# Autodesk Inventor assembly: Robot Assembly
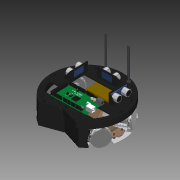
[picture p0: Inventor's stored thumbnail of the model, 180x180]
Saved by Autodesk Inventor 2015 (Build 190159000, 159)
## iProperties
Created: 2015-10-10
Part Number: Robot Assembly
Document SubType Name: Assembly
Designer: James
Mass: 1382.52 g
Surface Area: 3536.41 cm^2
Volume: 667.036 cm^3
Density: 2.07263 g/cm^3
Author: James
## Documents named in this file (21)
- C:\Users\James\Dropbox\Robotics 2016\Design\3D Printing\Robot Assembly.iam
- C:\Users\James\Dropbox\Robotics 2016\Design\3D Printing\Bottom Plate.ipt
- C:\Users\James\Dropbox\Robotics 2016\Design\3D Printing\Rod.ipt
- C:\Users\James\Dropbox\Robotics 2016\Design\3D Printing\Bottom Plate Standoff.ipt
- C:\Users\James\Dropbox\Robotics 2016\Design\3D Printing\Motor Mount Standoff.ipt
- C:\Users\James\Dropbox\Robotics 2016\Design\3D Printing\Motor Mount Bracket.ipt
- C:\Users\James\Dropbox\Robotics 2016\Design\3D Printing\Motor.ipt
- C:\Users\James\Dropbox\Robotics 2016\Design\3D Printing\Spacer 5.ipt
- C:\Users\James\Dropbox\Robotics 2016\Design\3D Printing\Veroboard Bottom Plate.ipt
- C:\Users\James\Dropbox\Robotics 2016\Design\3D Printing\Rod Spacer.ipt
- C:\Users\James\Dropbox\Robotics 2016\Design\3D Printing\Middle Plate.ipt
- C:\Users\James\Dropbox\Robotics 2016\Design\3D Printing\Nut Rod.ipt
- C:\Users\James\Dropbox\Robotics 2016\Design\3D Printing\Wheel.ipt
- C:\Users\James\Dropbox\Robotics 2016\Design\3D Printing\ArduinoMEGA2560.ipt
- C:\Users\James\Dropbox\Robotics 2016\Design\3D Printing\Verboard Middle Plate.ipt
- C:\Users\James\Dropbox\Robotics 2016\Design\3D Printing\M3 6mm screw.ipt
- C:\Users\James\Dropbox\Robotics 2016\Design\3D Printing\M3 hex nut.ipt
- C:\Users\James\Dropbox\Robotics 2016\Design\3D Printing\HC-SR04 Sonar.ipt
- C:\Users\James\Dropbox\Robotics 2016\Design\3D Printing\Battery.ipt
- C:\Users\James\Dropbox\Robotics 2016\Design\3D Printing\Spacer 25.ipt
- C:\Users\James\Dropbox\Robotics 2016\Design\3D Printing\Spacer 45.ipt
## Components (99 placed, 20 different names)
1. Bottom Plate:1 — Mate:2, Mate:3, Mate:5, Mate:6, Mate:9, Mate:12, Mate:13, Mate:14, Mate:15, Mate:16, Mate:17, Mate:18, Mate:19, Mate:20, Mate:21, Mate:22, Mate:23, Mate:48, Mate:49, Mate:50, Mate:51, Mate:52, Mate:53, Mate:54, Mate:55, Mate:56, Mate:57, Mate:58, Mate:59, Mate:60, Mate:61, Mate:62, Mate:63, Mate:64, Mate:65, Mate:66, Mate:67, Mate:68, Mate:69, Mate:70, Mate:71, Mate:72, Mate:73, Mate:74, Mate:75, Mate:153, Mate:154, Mate:155, Mate:156, Mate:157, Mate:158, Mate:159, Mate:160, Mate:161, Mate:162, Mate:163, Mate:164, Mate:165, Mate:166, Mate:167, Mate:168, Mate:169, Mate:170, Mate:171, Mate:172, Mate:173, Mate:174, Mate:175, Mate:176, Mate:177, Mate:178, Mate:179, Mate:180, Mate:381, Mate:382, Mate:385, Mate:386, Mate:387, Mate:388, Mate:389, Mate:390, Mate:443, Mate:444
2. Rod:2 — Mate:2, Mate:6, Mate:91, Mate:384
3. Rod:3 — Mate:3, Mate:5, Mate:90, Mate:383
4. Bottom Plate Standoff:1 — Mate:9, Mate:83
5. Motor Mount Standoff:1 — Mate:12, Mate:20, Mate:21, Mate:24, Mate:32, Mate:33
6. Motor Mount Standoff:2 — Mate:13, Mate:16, Mate:17, Mate:25, Mate:30, Mate:31
7. Motor Mount Standoff:3 — Mate:14, Mate:22, Mate:23, Mate:26, Mate:34, Mate:35
8. Motor Mount Standoff:4 — Mate:15, Mate:18, Mate:19, Mate:27, Mate:28, Mate:29
9. Motor Mount Bracket:1 — Mate:25, Mate:30, Mate:31, Mate:37, Mate:41, Mate:46
10. Motor Mount Bracket:2 — Mate:27, Mate:28, Mate:29, Mate:39, Mate:42, Mate:47
11. Motor Mount Bracket:3 — Mate:26, Mate:34, Mate:35, Mate:38, Mate:40, Mate:45
12. Motor Mount Bracket:4 — Mate:24, Mate:32, Mate:33, Mate:36, Mate:43, Mate:44
13. Motor:1 — Mate:36, Mate:43, Mate:44, Flush:4, Mate:97
14. Motor:2 — Mate:37, Mate:41, Mate:46, Flush:1, Mate:94
15. Motor:3 — Mate:38, Mate:40, Mate:45, Flush:3, Mate:96
16. Motor:4 — Mate:39, Mate:42, Mate:47, Flush:2, Mate:95
17. Spacer 5:1 — Mate:53, Mate:69, Mate:204
18. Spacer 5:2 — Mate:52, Mate:73, Mate:205
19. Spacer 5:3 — Mate:49, Mate:68, Mate:420
20. Spacer 5:4 — Mate:48, Mate:67, Mate:77, Mate:425
21. Spacer 5:5 — Mate:51, Mate:64, Mate:76, Mate:421
22. Spacer 5:6 — Mate:50, Mate:65, Mate:423
23. Spacer 5:7 — Mate:55, Mate:62, Mate:195
24. Spacer 5:8 — Mate:54, Mate:66, Mate:78, Mate:427
25. Spacer 5:9 — Mate:56, Mate:71, Mate:200
26. Spacer 5:10 — Mate:57, Mate:74, Mate:201
27. Spacer 5:11 — Mate:60, Mate:75, Mate:206
28. Spacer 5:12 — Mate:58, Mate:63, Mate:196
29. Spacer 5:13 — Mate:59, Mate:72, Mate:202
30. Spacer 5:14 — Mate:61, Mate:70, Mate:199
31. Veroboard Bottom Plate:1 — Mate:76, Mate:77, Mate:78, Mate:181, Mate:183, Mate:184, Mate:185, Mate:186, Mate:187, Mate:188, Mate:189, Mate:191, Mate:193, Mate:422, Mate:424, Mate:426, Mate:428
32. Rod Spacer:1 — Mate:382, Mate:383, Mate:385, Mate:391, Mate:395, Mate:396
33. Rod Spacer:2 — Mate:381, Mate:384, Mate:386, Mate:393, Mate:397
34. Middle Plate:1 — Mate:83, Mate:86, Mate:89, Mate:109, Mate:111, Mate:113, Mate:114, Mate:116, Mate:221, Mate:222, Mate:223, Mate:224, Mate:225, Mate:250, Mate:251, Mate:375, Mate:376, Mate:377, Mate:378, Mate:379, Mate:380, Mate:399, Mate:401, Mate:402, Mate:440, Mate:441, Mate:442
35. Nut Rod:1 — Mate:86, Mate:91
36. Nut Rod:4 — Mate:89, Mate:90
37. Wheel:1 — Flush:4, Mate:97
38. Wheel:2 — Flush:3, Mate:96
39. Wheel:3 — Flush:2, Mate:95
40. Wheel:4 — Flush:1, Mate:94
41. Spacer 5:15 — Mate:114, Mate:225, Mate:226, Mate:257
42. Spacer 5:17 — Mate:111, Mate:221, Mate:227, Mate:243
43. Spacer 5:20 — Mate:109, Mate:223, Mate:247
44. Spacer 5:22 — Mate:113, Mate:222, Mate:242
45. Spacer 5:23 — Mate:116, Mate:224, Mate:228, Mate:256
46. -  -:1 — Mate:226, Mate:227, Mate:228, Mate:229, Mate:230, Mate:231, Mate:232, Mate:233, Mate:234, Mate:235, Mate:236, Mate:237, Mate:238
47. Verboard Middle Plate:1 — Mate:429, Mate:430, Mate:431, Mate:432, Mate:433, Mate:434, Mate:435
48. M3 6mm screw:6 — Mate:153, Mate:165
49. M3 6mm screw:8 — Mate:154, Mate:167
50. M3 6mm screw:9 — Mate:155, Mate:168
51. M3 6mm screw:10 — Mate:156, Mate:170
52. M3 6mm screw:11 — Mate:157, Mate:166
53. M3 6mm screw:12 — Mate:158, Mate:171
54. M3 6mm screw:13 — Mate:159, Mate:172
55. M3 6mm screw:14 — Mate:160, Mate:169
56. M3 6mm screw:15 — Mate:161, Mate:173
57. M3 6mm screw:16 — Mate:162, Mate:174
58. M3 6mm screw:17 — Mate:163, Mate:175
59. M3 6mm screw:18 — Mate:164, Mate:176
60. M3 6mm screw:19 — Mate:177, Mate:179
61. M3 6mm screw:20 — Mate:178, Mate:180
62. M3 hex nut:1 — Mate:181, Mate:196
63. M3 hex nut:3 — Mate:183, Mate:204
64. M3 hex nut:4 — Mate:184, Mate:200
65. M3 hex nut:5 — Mate:185, Mate:202
66. M3 hex nut:6 — Mate:186, Mate:205
67. M3 hex nut:7 — Mate:188, Mate:206
68. M3 hex nut:8 — Mate:187, Mate:420
69. M3 hex nut:9 — Mate:189, Mate:195
70. M3 hex nut:11 — Mate:193, Mate:199
71. M3 hex nut:12 — Mate:191, Mate:201
72. M3 hex nut:15 — Mate:247, Mate:402
73. M3 hex nut:17 — Mate:242, Mate:401
74. M3 hex nut:21 — Mate:243, Mate:399
75. M3 6mm screw:21 — Mate:230, Mate:234
76. M3 6mm screw:22 — Mate:233, Mate:237
77. M3 6mm screw:23 — Mate:232, Mate:238
78. M3 6mm screw:24 — Mate:231, Mate:235
79. M3 6mm screw:25 — Mate:229, Mate:236
80. M3 hex nut:26 — Mate:251, Mate:256
81. M3 hex nut:27 — Mate:250, Mate:257
82. HC-SR04 Sonar:1 — Mate:375, Mate:376, Mate:377
83. HC-SR04 Sonar:2 — Mate:378, Mate:379, Mate:380
84. Battery:1 — Mate:395, Mate:396, Mate:397
85. M3 6mm screw:34 — Mate:387, Mate:389, Mate:394
86. M3 6mm screw:35 — Mate:388, Mate:390, Mate:392
87. M3 hex nut:32 — Mate:391, Mate:392
88. M3 hex nut:33 — Mate:393, Mate:394
89. Spacer 25:1 — Mate:427, Mate:428, Mate:430, Mate:439
90. Spacer 25:2 — Mate:425, Mate:426, Mate:431, Mate:438
91. Spacer 25:3 — Mate:423, Mate:424, Mate:437
92. Spacer 25:4 — Mate:421, Mate:422, Mate:429, Mate:436
93. M3 hex nut:34 — Mate:434, Mate:437
94. M3 hex nut:35 — Mate:435, Mate:439
95. M3 hex nut:36 — Mate:433, Mate:436
96. M3 hex nut:37 — Mate:432, Mate:438
97. HC-SR04 Sonar:3 — Mate:440, Mate:441, Mate:442
98. Spacer 45:1 — Mate:443, Mate:444
99. Spacer 45:2
## Relationships (213: Mate 209, Flush 4)
- Mate:2: Bottom Plate:1 ↔ Rod:2
- Mate:3: Bottom Plate:1 ↔ Rod:3
- Mate:5: Bottom Plate:1 ↔ Rod:3
- Mate:6: Bottom Plate:1 ↔ Rod:2
- Mate:9: Bottom Plate:1 ↔ Bottom Plate Standoff:1
- Mate:12: Bottom Plate:1 ↔ Motor Mount Standoff:1
- Mate:13: Bottom Plate:1 ↔ Motor Mount Standoff:2
- Mate:14: Bottom Plate:1 ↔ Motor Mount Standoff:3
- Mate:15: Bottom Plate:1 ↔ Motor Mount Standoff:4
- Mate:16: Bottom Plate:1 ↔ Motor Mount Standoff:2
- Mate:17: Bottom Plate:1 ↔ Motor Mount Standoff:2
- Mate:18: Bottom Plate:1 ↔ Motor Mount Standoff:4
- Mate:19: Bottom Plate:1 ↔ Motor Mount Standoff:4
- Mate:20: Bottom Plate:1 ↔ Motor Mount Standoff:1
- Mate:21: Bottom Plate:1 ↔ Motor Mount Standoff:1
- Mate:22: Bottom Plate:1 ↔ Motor Mount Standoff:3
- Mate:23: Bottom Plate:1 ↔ Motor Mount Standoff:3
- Mate:24: Motor Mount Standoff:1 ↔ Motor Mount Bracket:4
- Mate:25: Motor Mount Standoff:2 ↔ Motor Mount Bracket:1
- Mate:26: Motor Mount Standoff:3 ↔ Motor Mount Bracket:3
- Mate:27: Motor Mount Standoff:4 ↔ Motor Mount Bracket:2
- Mate:28: Motor Mount Standoff:4 ↔ Motor Mount Bracket:2
- Mate:29: Motor Mount Standoff:4 ↔ Motor Mount Bracket:2
- Mate:30: Motor Mount Standoff:2 ↔ Motor Mount Bracket:1
- Mate:31: Motor Mount Standoff:2 ↔ Motor Mount Bracket:1
- Mate:32: Motor Mount Standoff:1 ↔ Motor Mount Bracket:4
- Mate:33: Motor Mount Standoff:1 ↔ Motor Mount Bracket:4
- Mate:34: Motor Mount Standoff:3 ↔ Motor Mount Bracket:3
- Mate:35: Motor Mount Standoff:3 ↔ Motor Mount Bracket:3
- Mate:36: Motor Mount Bracket:4 ↔ Motor:1
- Mate:37: Motor Mount Bracket:1 ↔ Motor:2
- Mate:38: Motor Mount Bracket:3 ↔ Motor:3
- Mate:39: Motor Mount Bracket:2 ↔ Motor:4
- Mate:40: Motor Mount Bracket:3 ↔ Motor:3
- Mate:41: Motor Mount Bracket:1 ↔ Motor:2
- Mate:42: Motor Mount Bracket:2 ↔ Motor:4
- Mate:43: Motor Mount Bracket:4 ↔ Motor:1
- Mate:44: Motor Mount Bracket:4 ↔ Motor:1
- Mate:45: Motor Mount Bracket:3 ↔ Motor:3
- Mate:46: Motor Mount Bracket:1 ↔ Motor:2
- Mate:47: Motor Mount Bracket:2 ↔ Motor:4
- Mate:48: Bottom Plate:1 ↔ Spacer 5:4
- Mate:49: Bottom Plate:1 ↔ Spacer 5:3
- Mate:50: Bottom Plate:1 ↔ Spacer 5:6
- Mate:51: Bottom Plate:1 ↔ Spacer 5:5
- Mate:52: Bottom Plate:1 ↔ Spacer 5:2
- Mate:53: Bottom Plate:1 ↔ Spacer 5:1
- Mate:54: Bottom Plate:1 ↔ Spacer 5:8
- Mate:55: Bottom Plate:1 ↔ Spacer 5:7
- Mate:56: Bottom Plate:1 ↔ Spacer 5:9
- Mate:57: Bottom Plate:1 ↔ Spacer 5:10
- Mate:58: Bottom Plate:1 ↔ Spacer 5:12
- Mate:59: Bottom Plate:1 ↔ Spacer 5:13
- Mate:60: Bottom Plate:1 ↔ Spacer 5:11
- Mate:61: Bottom Plate:1 ↔ Spacer 5:14
- Mate:62: Bottom Plate:1 ↔ Spacer 5:7
- Mate:63: Bottom Plate:1 ↔ Spacer 5:12
- Mate:64: Bottom Plate:1 ↔ Spacer 5:5
- Mate:65: Bottom Plate:1 ↔ Spacer 5:6
- Mate:66: Bottom Plate:1 ↔ Spacer 5:8
- Mate:67: Bottom Plate:1 ↔ Spacer 5:4
- Mate:68: Bottom Plate:1 ↔ Spacer 5:3
- Mate:69: Bottom Plate:1 ↔ Spacer 5:1
- Mate:70: Bottom Plate:1 ↔ Spacer 5:14
- Mate:71: Bottom Plate:1 ↔ Spacer 5:9
- Mate:72: Bottom Plate:1 ↔ Spacer 5:13
- Mate:73: Bottom Plate:1 ↔ Spacer 5:2
- Mate:74: Bottom Plate:1 ↔ Spacer 5:10
- Mate:75: Bottom Plate:1 ↔ Spacer 5:11
- Mate:76: Spacer 5:5 ↔ Veroboard Bottom Plate:1
- Mate:77: Spacer 5:4 ↔ Veroboard Bottom Plate:1
- Mate:78: Spacer 5:8 ↔ Veroboard Bottom Plate:1
- Mate:83: Bottom Plate Standoff:1 ↔ Middle Plate:1
- Mate:86: Middle Plate:1 ↔ Nut Rod:1
- Mate:89: Middle Plate:1 ↔ Nut Rod:4
- Mate:90: Rod:3 ↔ Nut Rod:4
- Mate:91: Rod:2 ↔ Nut Rod:1
- Flush:1: Motor:2 ↔ Wheel:4
- Mate:94: Motor:2 ↔ Wheel:4
- Flush:2: Motor:4 ↔ Wheel:3
- Mate:95: Motor:4 ↔ Wheel:3
- Flush:3: Motor:3 ↔ Wheel:2
- Mate:96: Motor:3 ↔ Wheel:2
- Flush:4: Motor:1 ↔ Wheel:1
- Mate:97: Motor:1 ↔ Wheel:1
- Mate:109: Middle Plate:1 ↔ Spacer 5:20
- Mate:111: Middle Plate:1 ↔ Spacer 5:17
- Mate:113: Middle Plate:1 ↔ Spacer 5:22
- Mate:114: Middle Plate:1 ↔ Spacer 5:15
- Mate:116: Middle Plate:1 ↔ Spacer 5:23
- Mate:153: Bottom Plate:1 ↔ M3 6mm screw:6
- Mate:154: Bottom Plate:1 ↔ M3 6mm screw:8
- Mate:155: Bottom Plate:1 ↔ M3 6mm screw:9
- Mate:156: Bottom Plate:1 ↔ M3 6mm screw:10
- Mate:157: Bottom Plate:1 ↔ M3 6mm screw:11
- Mate:158: Bottom Plate:1 ↔ M3 6mm screw:12
- Mate:159: Bottom Plate:1 ↔ M3 6mm screw:13
- Mate:160: Bottom Plate:1 ↔ M3 6mm screw:14
- Mate:161: Bottom Plate:1 ↔ M3 6mm screw:15
- Mate:162: Bottom Plate:1 ↔ M3 6mm screw:16
- Mate:163: Bottom Plate:1 ↔ M3 6mm screw:17
- Mate:164: Bottom Plate:1 ↔ M3 6mm screw:18
- Mate:165: Bottom Plate:1 ↔ M3 6mm screw:6
- Mate:166: Bottom Plate:1 ↔ M3 6mm screw:11
- Mate:167: Bottom Plate:1 ↔ M3 6mm screw:8
- Mate:168: Bottom Plate:1 ↔ M3 6mm screw:9
- Mate:169: Bottom Plate:1 ↔ M3 6mm screw:14
- Mate:170: Bottom Plate:1 ↔ M3 6mm screw:10
- Mate:171: Bottom Plate:1 ↔ M3 6mm screw:12
- Mate:172: Bottom Plate:1 ↔ M3 6mm screw:13
- Mate:173: Bottom Plate:1 ↔ M3 6mm screw:15
- Mate:174: Bottom Plate:1 ↔ M3 6mm screw:16
- Mate:175: Bottom Plate:1 ↔ M3 6mm screw:17
- Mate:176: Bottom Plate:1 ↔ M3 6mm screw:18
- Mate:177: Bottom Plate:1 ↔ M3 6mm screw:19
- Mate:178: Bottom Plate:1 ↔ M3 6mm screw:20
- Mate:179: Bottom Plate:1 ↔ M3 6mm screw:19
- Mate:180: Bottom Plate:1 ↔ M3 6mm screw:20
- Mate:181: Veroboard Bottom Plate:1 ↔ M3 hex nut:1
- Mate:183: Veroboard Bottom Plate:1 ↔ M3 hex nut:3
- Mate:184: Veroboard Bottom Plate:1 ↔ M3 hex nut:4
- Mate:185: Veroboard Bottom Plate:1 ↔ M3 hex nut:5
- Mate:186: Veroboard Bottom Plate:1 ↔ M3 hex nut:6
- Mate:187: Veroboard Bottom Plate:1 ↔ M3 hex nut:8
- Mate:188: Veroboard Bottom Plate:1 ↔ M3 hex nut:7
- Mate:189: Veroboard Bottom Plate:1 ↔ M3 hex nut:9
- Mate:191: Veroboard Bottom Plate:1 ↔ M3 hex nut:12
- Mate:193: Veroboard Bottom Plate:1 ↔ M3 hex nut:11
- Mate:195: Spacer 5:7 ↔ M3 hex nut:9
- Mate:196: Spacer 5:12 ↔ M3 hex nut:1
- Mate:199: Spacer 5:14 ↔ M3 hex nut:11
- Mate:200: Spacer 5:9 ↔ M3 hex nut:4
- Mate:201: Spacer 5:10 ↔ M3 hex nut:12
- Mate:202: Spacer 5:13 ↔ M3 hex nut:5
- Mate:204: Spacer 5:1 ↔ M3 hex nut:3
- Mate:205: Spacer 5:2 ↔ M3 hex nut:6
- Mate:206: Spacer 5:11 ↔ M3 hex nut:7
- Mate:221: Middle Plate:1 ↔ Spacer 5:17
- Mate:222: Middle Plate:1 ↔ Spacer 5:22
- Mate:223: Middle Plate:1 ↔ Spacer 5:20
- Mate:224: Middle Plate:1 ↔ Spacer 5:23
- Mate:225: Middle Plate:1 ↔ Spacer 5:15
- Mate:226: Spacer 5:15 ↔ -  -:1
- Mate:227: Spacer 5:17 ↔ -  -:1
- Mate:228: Spacer 5:23 ↔ -  -:1
- Mate:229: -  -:1 ↔ M3 6mm screw:25
- Mate:230: -  -:1 ↔ M3 6mm screw:21
- Mate:231: -  -:1 ↔ M3 6mm screw:24
- Mate:232: -  -:1 ↔ M3 6mm screw:23
- Mate:233: -  -:1 ↔ M3 6mm screw:22
- Mate:234: -  -:1 ↔ M3 6mm screw:21
- Mate:235: -  -:1 ↔ M3 6mm screw:24
- Mate:236: -  -:1 ↔ M3 6mm screw:25
- Mate:237: -  -:1 ↔ M3 6mm screw:22
- Mate:238: -  -:1 ↔ M3 6mm screw:23
- Mate:242: Spacer 5:22 ↔ M3 hex nut:17
- Mate:243: Spacer 5:17 ↔ M3 hex nut:21
- Mate:247: Spacer 5:20 ↔ M3 hex nut:15
- Mate:250: Middle Plate:1 ↔ M3 hex nut:27
- Mate:251: Middle Plate:1 ↔ M3 hex nut:26
- Mate:256: Spacer 5:23 ↔ M3 hex nut:26
- Mate:257: Spacer 5:15 ↔ M3 hex nut:27
- Mate:375 (1 mm): Middle Plate:1 ↔ HC-SR04 Sonar:1
- Mate:376: Middle Plate:1 ↔ HC-SR04 Sonar:1
- Mate:377: Middle Plate:1 ↔ HC-SR04 Sonar:1
- Mate:378: Middle Plate:1 ↔ HC-SR04 Sonar:2
- Mate:379: Middle Plate:1 ↔ HC-SR04 Sonar:2
- Mate:380: Middle Plate:1 ↔ HC-SR04 Sonar:2
- Mate:381: Bottom Plate:1 ↔ Rod Spacer:2
- Mate:382: Bottom Plate:1 ↔ Rod Spacer:1
- Mate:383: Rod:3 ↔ Rod Spacer:1
- Mate:384: Rod:2 ↔ Rod Spacer:2
- Mate:385: Bottom Plate:1 ↔ Rod Spacer:1
- Mate:386: Bottom Plate:1 ↔ Rod Spacer:2
- Mate:387: Bottom Plate:1 ↔ M3 6mm screw:34
- Mate:388: Bottom Plate:1 ↔ M3 6mm screw:35
- Mate:389: Bottom Plate:1 ↔ M3 6mm screw:34
- Mate:390: Bottom Plate:1 ↔ M3 6mm screw:35
- Mate:391: Rod Spacer:1 ↔ M3 hex nut:32
- Mate:392: M3 6mm screw:35 ↔ M3 hex nut:32
- Mate:393: Rod Spacer:2 ↔ M3 hex nut:33
- Mate:394: M3 6mm screw:34 ↔ M3 hex nut:33
- Mate:395: Rod Spacer:1 ↔ Battery:1
- Mate:396 (7 mm): Rod Spacer:1 ↔ Battery:1
- Mate:397 (7 mm): Rod Spacer:2 ↔ Battery:1
- Mate:399: Middle Plate:1 ↔ M3 hex nut:21
- Mate:401: Middle Plate:1 ↔ M3 hex nut:17
- Mate:402: Middle Plate:1 ↔ M3 hex nut:15
- Mate:420: Spacer 5:3 ↔ M3 hex nut:8
- Mate:421: Spacer 5:5 ↔ Spacer 25:4
- Mate:422: Veroboard Bottom Plate:1 ↔ Spacer 25:4
- Mate:423: Spacer 5:6 ↔ Spacer 25:3
- Mate:424: Veroboard Bottom Plate:1 ↔ Spacer 25:3
- Mate:425: Spacer 5:4 ↔ Spacer 25:2
- Mate:426: Veroboard Bottom Plate:1 ↔ Spacer 25:2
- Mate:427: Spacer 5:8 ↔ Spacer 25:1
- Mate:428: Veroboard Bottom Plate:1 ↔ Spacer 25:1
- Mate:429: Verboard Middle Plate:1 ↔ Spacer 25:4
- Mate:430: Verboard Middle Plate:1 ↔ Spacer 25:1
- Mate:431: Verboard Middle Plate:1 ↔ Spacer 25:2
- Mate:432: Verboard Middle Plate:1 ↔ M3 hex nut:37
- Mate:433: Verboard Middle Plate:1 ↔ M3 hex nut:36
- Mate:434: Verboard Middle Plate:1 ↔ M3 hex nut:34
- Mate:435: Verboard Middle Plate:1 ↔ M3 hex nut:35
- Mate:436: Spacer 25:4 ↔ M3 hex nut:36
- Mate:437: Spacer 25:3 ↔ M3 hex nut:34
- Mate:438: Spacer 25:2 ↔ M3 hex nut:37
- Mate:439: Spacer 25:1 ↔ M3 hex nut:35
- Mate:440 (1 mm): Middle Plate:1 ↔ HC-SR04 Sonar:3
- Mate:441: Middle Plate:1 ↔ HC-SR04 Sonar:3
- Mate:442: Middle Plate:1 ↔ HC-SR04 Sonar:3
- Mate:443: Bottom Plate:1 ↔ Spacer 45:1
- Mate:444: Bottom Plate:1 ↔ Spacer 45:1
